# Autodesk Inventor assembly: Assembly1
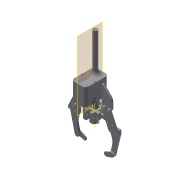
[picture p0: Inventor's stored thumbnail of the model, 180x180]
Saved by Autodesk Inventor 2018 (Build 220112000, 112)
## iProperties
Created: 2018-05-21
Part Number: Assembly1
Document SubType Name: Assembly
Designer: Bardo91
Author: Bardo91
## Documents named in this file (8)
- E:\programming\hecatonquiros\cad_models\tools\gripper\serial_model_0dof\Assembly1.iam
- E:\programming\hecatonquiros\cad_models\tools\gripper\serial_model_0dof\core_attachment.ipt
- E:\programming\hecatonquiros\cad_models\tools\gripper\serial_model_0dof\case_core.ipt
- E:\programming\hecatonquiros\cad_models\tools\gripper\serial_model_0dof\bar.ipt
- E:\programming\hecatonquiros\cad_models\tools\gripper\serial_model_0dof\gripper.ipt
- E:\programming\hecatonquiros\cad_models\tools\gripper\serial_model_0dof\ScrewActuatorGripper.ipt
- E:\programming\hecatonquiros\cad_models\tools\gripper\serial_model_0dof\ScrewActuatorGripperCenter.ipt
- E:\programming\hecatonquiros\cad_models\tools\gripper\serial_model_0dof\barMini.ipt
## Components (12 placed, 7 different names)
1. core_attachment:1 — Mate:1, Mate:2, Mate:3, Mate:10, Mate:11, Mate:17, Mate:18, Mate:24, Mate:25, Mate:39, Mate:40, Mate:41, Mate:42
2. case_core:1 — Mate:1, Mate:2, Mate:3
3. bar:2 — Mate:11, Mate:37, Mate:39, Mate:44
4. bar:4 — Mate:10, Mate:40, Mate:43, Mate:45
5. gripper:1 — Mate:43, Mate:44
6. ScrewActuatorGripper:1 — Mate:17, Mate:18, Mate:19
7. ScrewActuatorGripperCenter:1 — Mate:19, Mate:33, Mate:35
8. barMini:1 — Mate:35, Mate:37, Mate:45
9. barMini:2 — Mate:33, Mate:38, Mate:48
10. bar:5 — Mate:25, Mate:38, Mate:41, Mate:46, Mate:48
11. bar:6 — Mate:24, Mate:42, Mate:47
12. gripper:2 — Mate:46, Mate:47
## Relationships (24: Mate 24)
- Mate:1: core_attachment:1 ↔ case_core:1
- Mate:2: core_attachment:1 ↔ case_core:1
- Mate:3: core_attachment:1 ↔ case_core:1
- Mate:10: core_attachment:1 ↔ bar:4
- Mate:11: core_attachment:1 ↔ bar:2
- Mate:17: core_attachment:1 ↔ ScrewActuatorGripper:1
- Mate:18: core_attachment:1 ↔ ScrewActuatorGripper:1
- Mate:19: ScrewActuatorGripper:1 ↔ ScrewActuatorGripperCenter:1
- Mate:24: core_attachment:1 ↔ bar:6
- Mate:25: core_attachment:1 ↔ bar:5
- Mate:33: ScrewActuatorGripperCenter:1 ↔ barMini:2
- Mate:35: ScrewActuatorGripperCenter:1 ↔ barMini:1
- Mate:37: bar:2 ↔ barMini:1
- Mate:38: barMini:2 ↔ bar:5
- Mate:39: core_attachment:1 ↔ bar:2
- Mate:40: core_attachment:1 ↔ bar:4
- Mate:41: core_attachment:1 ↔ bar:5
- Mate:42: core_attachment:1 ↔ bar:6
- Mate:43: bar:4 ↔ gripper:1
- Mate:44: bar:2 ↔ gripper:1
- Mate:45: bar:4 ↔ barMini:1
- Mate:46: bar:5 ↔ gripper:2
- Mate:47: bar:6 ↔ gripper:2
- Mate:48: barMini:2 ↔ bar:5
